# Autodesk Inventor assembly: ASM_Vial_and_Header
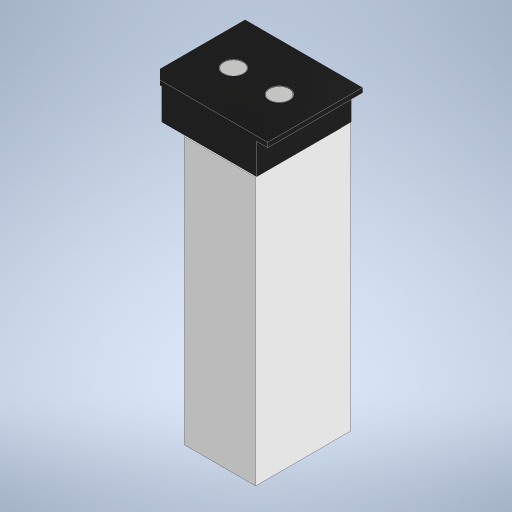
[picture p0: Inventor's stored thumbnail of the model, 512x512]
Saved by Autodesk Inventor 2024 (Build 280153000, 153)
## iProperties
Created: 2024-04-23
Part Number: ASM_Vial_and_Header
Document SubType Name: Assembly
Designer: jamha
Author: jamha
## Documents named in this file (5)
- C:\Users\jamha\OneDrive - The University of Texas at Dallas\SD - TEAM 1830\Final Deliverable\CAD Final Deliverable\Sample Tray Full Assembly\ASM_Vial_and_Header.iam
- C:\Users\jamha\OneDrive - The University of Texas at Dallas\SD - TEAM 1830\Final Deliverable\CAD Final Deliverable\Sample Tray Full Assembly\IPT_Custom_Made_Vial_Sleeve.ipt
- C:\Users\jamha\OneDrive - The University of Texas at Dallas\SD - TEAM 1830\Final Deliverable\CAD Final Deliverable\Sample Tray Full Assembly\IPT_Header.ipt
- C:\Users\jamha\OneDrive - The University of Texas at Dallas\SD - TEAM 1830\Final Deliverable\CAD Final Deliverable\Sample Tray Full Assembly\IPT_Neodymium_Magnet.ipt
- C:\Users\jamha\OneDrive - The University of Texas at Dallas\SD - TEAM 1830\Final Deliverable\CAD Final Deliverable\Sample Tray Full Assembly\IPT_Threaded_Insert.ipt
## Components (5 placed, 4 different names)
1. IPT_Custom_Made_Vial_Sleeve:1 — Mate:1, Angle:1, Mate:6
2. IPT_Header:1 — Mate:1, Angle:1, Mate:2, Mate:3, Mate:4, Mate:5, Mate:6, Mate:7, Flush:1
3. IPT_Neodymium_Magnet:1 — Mate:2, Mate:3
4. IPT_Neodymium_Magnet:2 — Mate:4, Mate:5
5. IPT_Threaded_Insert:1 — Mate:7, Flush:1
## Relationships (9: Mate 7, Angle 1, Flush 1)
- Mate:1: IPT_Custom_Made_Vial_Sleeve:1 ↔ IPT_Header:1
- Angle:1 (0 deg): IPT_Custom_Made_Vial_Sleeve:1 ↔ IPT_Header:1
- Mate:2: IPT_Header:1 ↔ IPT_Neodymium_Magnet:1
- Mate:3: IPT_Header:1 ↔ IPT_Neodymium_Magnet:1
- Mate:4: IPT_Header:1 ↔ IPT_Neodymium_Magnet:2
- Mate:5: IPT_Header:1 ↔ IPT_Neodymium_Magnet:2
- Mate:6: IPT_Custom_Made_Vial_Sleeve:1 ↔ IPT_Header:1
- Mate:7: IPT_Header:1 ↔ IPT_Threaded_Insert:1
- Flush:1: IPT_Header:1 ↔ IPT_Threaded_Insert:1
